# Autodesk Inventor assembly: tren
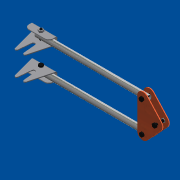
[picture p0: Inventor's stored thumbnail of the model, 180x180]
Saved by Autodesk Inventor 2016 (Build 200138000, 138)
## iProperties
Created: 2017-05-13
Part Number: tren
Document SubType Name: Assembly
Designer: Gian
Author: Gian
## Documents named in this file (6)
- C:\Users\Gian\Desktop\Pedalazo\002_Diseño\Version_001\tren.iam
- C:\Users\Gian\Desktop\Pedalazo\002_Diseño\Version_001\Tubo_conexion.ipt
- C:\Users\Gian\Desktop\Pedalazo\002_Diseño\Version_001\perno_38.ipt
- C:\Users\Gian\Desktop\Pedalazo\002_Diseño\Version_001\Conexion_eje.ipt
- C:\Users\Gian\Desktop\Pedalazo\002_Diseño\Version_001\Conexion_Rueda2.ipt
- C:\Users\Gian\Desktop\Pedalazo\002_Diseño\Version_001\Tuerca.ipt
## Components (16 placed, 5 different names)
1. Tubo_conexion:1 — Cylindrical:2, Flush:2, Cylindrical:4
2. Tubo_conexion:2 — Flush:2, Cylindrical:3
3. perno_38:1 — Cylindrical:11, Cylindrical:13
4. perno_38:2 — Cylindrical:7, Cylindrical:14
5. perno_38:3 — Cylindrical:8, Cylindrical:12
6. Conexion_eje:3 — Mate:1, Flush:1, Cylindrical:1
7. Conexion_eje:4 — Mate:1, Flush:1, Cylindrical:1, Cylindrical:2, Cylindrical:3, Cylindrical:7, Cylindrical:8, Flush:5, Cylindrical:11, Mate:2
8. Conexion_Rueda2:1 — Cylindrical:4, Flush:3, Flush:4, Cylindrical:6
9. Conexion_Rueda2:3 — Flush:3, Flush:4, Cylindrical:5, Flush:5
10. perno_38:4 — Cylindrical:6, Cylindrical:9
11. perno_38:5 — Cylindrical:5, Cylindrical:10
12. Tuerca:1 — Cylindrical:14
13. Tuerca:2 — Cylindrical:9
14. Tuerca:3 — Cylindrical:10
15. Tuerca:4 — Cylindrical:12
16. Tuerca:5 — Cylindrical:13
## Relationships (22: CylindricalJoint 14, Flush 5, Mate 2, Angle 1)
- Mate:1 (20 mm): Conexion_eje:3 ↔ Conexion_eje:4
- Flush:1: Conexion_eje:3 ↔ Conexion_eje:4
- Cylindrical:1: Conexion_eje:3 ↔ Conexion_eje:4
- Cylindrical:2: Tubo_conexion:1 ↔ Conexion_eje:4
- Flush:2: Tubo_conexion:1 ↔ Tubo_conexion:2
- Cylindrical:3: Tubo_conexion:2 ↔ Conexion_eje:4
- Cylindrical:4: Tubo_conexion:1 ↔ Conexion_Rueda2:1
- Flush:3: Conexion_Rueda2:1 ↔ Conexion_Rueda2:3
- Flush:4: Conexion_Rueda2:1 ↔ Conexion_Rueda2:3
- Cylindrical:5: Conexion_Rueda2:3 ↔ perno_38:5
- Cylindrical:6: Conexion_Rueda2:1 ↔ perno_38:4
- Cylindrical:7: perno_38:2 ↔ Conexion_eje:4
- Cylindrical:8: perno_38:3 ↔ Conexion_eje:4
- Cylindrical:9: perno_38:4 ↔ Tuerca:2
- Cylindrical:10: perno_38:5 ↔ Tuerca:3
- Flush:5: Conexion_eje:4 ↔ Conexion_Rueda2:3
- Cylindrical:11: perno_38:1 ↔ Conexion_eje:4
- Cylindrical:12: perno_38:3 ↔ Tuerca:4
- Cylindrical:13: perno_38:1 ↔ Tuerca:5
- Cylindrical:14: perno_38:2 ↔ Tuerca:1
- Mate:2: Conexion_eje:4
- Angle:1 (0 deg)
